# Autodesk Inventor assembly: LegAnkleUnitBasis
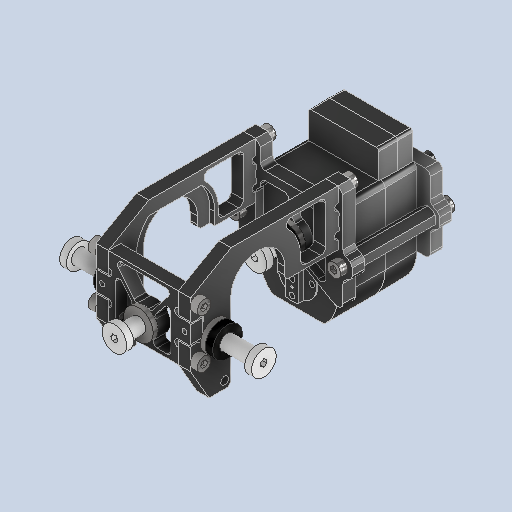
[picture p0: Inventor's stored thumbnail of the model, 512x512]
Saved by Autodesk Inventor 2024.2 (Build 282272000, 272)
## iProperties
Created: 2024-01-08
Part Number: LegAnkleUnitBasis
Document SubType Name: Assembly
Designer: Masato Kubotera
Mass: 189.091 g
Surface Area: 355.718 cm^2
Volume: 76.2964 cm^3
Density: 2.47837 g/cm^3
Author: Masato Kubotera
## Documents named in this file (9)
- C:\Users\masato\OneDrive - Chiba Institute of Technology\CIT Brains\RoboCup2024\Mechanic\SUSTAINA-OP2\NativeFiles\Boby\LowerLimb\Legs\LegBases\LegAnkleUnitBasis.iam
- C:\Users\masato\OneDrive - Chiba Institute of Technology\CIT Brains\RoboCup2024\Mechanic\SUSTAINA-OP2\NativeFiles\Boby\COTS\Actuators\PMX-SCR-5203HV.ipt
- C:\Users\masato\OneDrive - Chiba Institute of Technology\CIT Brains\RoboCup2024\Mechanic\SUSTAINA-OP2\NativeFiles\Boby\COTS\Screws\CapScrew\FC-2620EB.ipt
- C:\Users\masato\OneDrive - Chiba Institute of Technology\CIT Brains\RoboCup2024\Mechanic\SUSTAINA-OP2\NativeFiles\Boby\LowerLimb\Legs\LegBases\LegBaseUnitBasis.iam
- C:\Users\masato\OneDrive - Chiba Institute of Technology\CIT Brains\RoboCup2024\Mechanic\SUSTAINA-OP2\NativeFiles\Boby\COTS\Washers\Metal\UUW-0412-20H.ipt
- C:\Users\masato\OneDrive - Chiba Institute of Technology\CIT Brains\RoboCup2024\Mechanic\SUSTAINA-OP2\NativeFiles\Boby\COTS\Screws\ScrewsWithShoulder\DBSY4-7-5.ipt
- C:\Users\masato\OneDrive - Chiba Institute of Technology\CIT Brains\RoboCup2024\Mechanic\SUSTAINA-OP2\NativeFiles\Boby\LowerLimb\Legs\LegBases\LegBaseBackFrame.ipt
- C:\Users\masato\OneDrive - Chiba Institute of Technology\CIT Brains\RoboCup2024\Mechanic\SUSTAINA-OP2\NativeFiles\Boby\COTS\Screws\CapScrew\UC-0310.ipt
- C:\Users\masato\OneDrive - Chiba Institute of Technology\CIT Brains\RoboCup2024\Mechanic\SUSTAINA-OP2\NativeFiles\Boby\COTS\Spacers\ABLSBF6-32_5-M3-N3.ipt
## Components (11 placed, 8 different names)
1. LegBaseUnitBasis:1 [sub-assembly] — Flush:1, Flush:2, Flush:3, Insert:8, Insert:17, Insert:18
2. LegBaseBackFrame:1
3. PMX-SCR-5203HV:2
4. FC-2620EB:2
5. FC-2620EB:3
6. UC-0310:1
7. UC-0310:2
8. DBSY4-7-5:1
9. ABLSBF6-32_5-M3-N3:2 — Insert:17, Angle:1
10. ABLSBF6-32_5-M3-N3:1 — Insert:18, Angle:2
11. UUW-0412-20H:1 — Insert:8
## Relationships (17: Insert 12, Flush 3, Angle 2)
- Flush:1: LegBaseUnitBasis:1
- Flush:2: LegBaseUnitBasis:1
- Flush:3: LegBaseUnitBasis:1
- [Insert]: DBSY4-7-5:1 ↔ UUW-0412-20H:1
- Insert:8: LegBaseUnitBasis:1 ↔ UUW-0412-20H:1
- [Insert]: LegBaseBackFrame:1 ↔ PMX-SCR-5203HV:2
- [Insert]: LegBaseBackFrame:1 ↔ PMX-SCR-5203HV:2
- [Insert]: LegBaseBackFrame:1 ↔ FC-2620EB:2
- [Insert]: LegBaseBackFrame:1 ↔ FC-2620EB:3
- [Insert]: LegBaseBackFrame:1 ↔ ABLSBF6-32_5-M3-N3:2
- [Insert]: LegBaseBackFrame:1 ↔ ABLSBF6-32_5-M3-N3:1
- [Insert]: LegBaseBackFrame:1 ↔ UC-0310:1
- [Insert]: LegBaseBackFrame:1 ↔ UC-0310:2
- Insert:17: LegBaseUnitBasis:1 ↔ ABLSBF6-32_5-M3-N3:2
- Insert:18: LegBaseUnitBasis:1 ↔ ABLSBF6-32_5-M3-N3:1
- Angle:1 (0 deg): ABLSBF6-32_5-M3-N3:2
- Angle:2 (0 deg): ABLSBF6-32_5-M3-N3:1
## Named parameters: d64_d62 = 0 mm, d66_d57 = 0 mm, d67_d58 = 0 mm, d68_d59 = 0 mm, d69_d60 = 0 mm
